# Autodesk Inventor assembly: biggearsmallgearBOTTOMSPACER
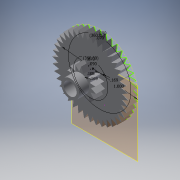
[picture p0: Inventor's stored thumbnail of the model, 180x180]
Saved by Autodesk Inventor 2018.3 (Build 223284000, 284)
## iProperties
Created: 2019-03-12
Part Number: biggearsmallgearBOTTOMSPACER
Document SubType Name: Assembly
Designer: F8PLTW
Author: F8PLTW
## Documents named in this file (3)
- D:\biggearsmallgearBOTTOMSPACER.iam
- D:\biggearsmallgearNOSPACER.iam
- D:\phonecasespacer.ipt
## Components (2 placed, 2 different names)
1. biggearsmallgearNOSPACER:1 [sub-assembly] — Mate:1, Mate:2
2. phonecasespacer:1 — Mate:1, Mate:2
## Relationships (2: Mate 2)
- Mate:1: biggearsmallgearNOSPACER:1 ↔ phonecasespacer:1
- Mate:2: biggearsmallgearNOSPACER:1 ↔ phonecasespacer:1
